# Autodesk Inventor assembly: Sorting Assembly
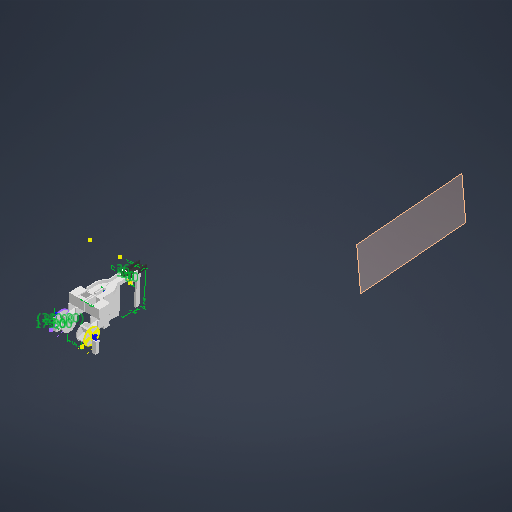
[picture p0: Inventor's stored thumbnail of the model, 512x512]
Saved by Autodesk Inventor 2026.2 (Build 302298000, 298)
## iProperties
Created: 2026-02-23
Part Number: Sorting Assembly
Document SubType Name: Assembly
Designer: danda
Author: danda
## Documents named in this file (17)
- C:\Users\danda\BOM-project\Project\CAD\sorting\Sorting Assembly.iam
- C:\Users\danda\BOM-project\Project\CAD\sorting\stand.ipt
- C:\Users\danda\BOM-project\Project\CAD\sorting\stand2.ipt
- C:\Users\danda\BOM-project\Project\CAD\sorting\inslide.ipt
- C:\Users\danda\BOM-project\Project\CAD\sorting\Towerpro Micro Servo 9g\Towerpro Micro Servo 9g\Towerpro Micro Servo 9g.ipt
- C:\Users\danda\BOM-project\Project\CAD\sorting\motorstand2.ipt
- C:\Users\danda\BOM-project\Project\CAD\sorting\gate2.ipt
- C:\Users\danda\BOM-project\Project\CAD\sorting\wheel.ipt
- C:\Users\danda\BOM-project\Project\CAD\sorting\motorwheelstand.ipt
- C:\Users\danda\BOM-project\Project\CAD\sorting\newmiddle.ipt
- C:\Users\danda\BOM-project\Project\CAD\sorting\leftcollection.ipt
- C:\Users\danda\BOM-project\Project\CAD\sorting\rightcollection.ipt
- C:\Users\danda\Downloads\ir-sensor-7.snapshot.2\Assembly2.iam
- C:\Users\danda\BOM-project\Project\CAD\sorting\wheel_MIR.ipt
- C:\Users\danda\BOM-project\Project\CAD\sorting\Towerpro Micro Servo 9g\Towerpro Micro Servo 9g\Towerpro Micro Servo 9g_MIR.ipt
- C:\Users\danda\BOM-project\Project\CAD\sorting\motorwheelstand_MIR.ipt
- C:\Users\danda\BOM-project\Project\CAD\Not needed\outstorage.ipt
## Components (18 placed, 16 different names)
1. stand:1 — Flush:8, Mate:30, Mate:73, Flush:40, Flush:42
2. stand2:1 — Mate:17, Mate:18, Mate:30, Mate:31, Mate:32, Flush:13
3. inslide:1 — Flush:8, Mate:17, Mate:18, Mate:31, Mate:32, Flush:13, Flush:34, Flush:35, Mate:67, Mate:68, Mate:71, Mate:72
4. motorstand2:1 — Mate:21, Mate:69, Mate:70, Flush:40, Flush:42, Flush:43, Flush:51
5. Towerpro Micro Servo 9g:2 — Mate:21, Mate:69, Mate:70, Insert:5
6. gate2:1 — Insert:5
7. wheel:1 — Insert:3, Mate:79, Flush:48
8. Towerpro Micro Servo 9g:4 — Mate:61, Mate:62, Mate:63, Insert:3
9. motorwheelstand:1 — Mate:61, Mate:62, Mate:63, Flush:50, Flush:51
10. newmiddle:1 — Flush:34, Flush:35, Mate:65, Flush:36, Flush:37, Mate:66, Flush:38, Flush:39, Mate:71, Mate:73, Flush:43
11. leftcollection:1 — Mate:66, Flush:38, Flush:39, Flush:41, Mate:77, Flush:44, Flush:45
12. rightcollection:1 — Mate:65, Flush:36, Flush:37, Flush:46, Flush:47, Mate:78
13. Assembly2:1 [sub-assembly] — Mate:67, Mate:68, Mate:72
14. wheel_MIR:1 — Insert:4, Mate:80, Flush:49
15. Towerpro Micro Servo 9g_MIR:1 — Insert:4, Mate:74, Mate:75, Mate:76
16. motorwheelstand_MIR:1 — Mate:74, Mate:75, Mate:76, Flush:50
17. outstorage:1 — Flush:46, Flush:47, Mate:78, Mate:80, Flush:49
18. outstorage:2 — Mate:77, Flush:44, Flush:45, Mate:79, Flush:48
## Relationships (48: Mate 25, Flush 20, Insert 3)
- Flush:8: stand:1 ↔ inslide:1
- Mate:17: stand2:1 ↔ inslide:1
- Mate:18: stand2:1 ↔ inslide:1
- Mate:21: motorstand2:1 ↔ Towerpro Micro Servo 9g:2
- Mate:30 (85 mm): stand:1 ↔ stand2:1
- Mate:31: stand2:1 ↔ inslide:1
- Mate:32: stand2:1 ↔ inslide:1
- Flush:13: stand2:1 ↔ inslide:1
- Mate:61: Towerpro Micro Servo 9g:4 ↔ motorwheelstand:1
- Mate:62: Towerpro Micro Servo 9g:4 ↔ motorwheelstand:1
- Mate:63: Towerpro Micro Servo 9g:4 ↔ motorwheelstand:1
- Flush:34: inslide:1 ↔ newmiddle:1
- Flush:35: inslide:1 ↔ newmiddle:1
- Mate:65: newmiddle:1 ↔ rightcollection:1
- Flush:36: newmiddle:1 ↔ rightcollection:1
- Flush:37: newmiddle:1 ↔ rightcollection:1
- Mate:66: newmiddle:1 ↔ leftcollection:1
- Flush:38: newmiddle:1 ↔ leftcollection:1
- Flush:39: newmiddle:1 ↔ leftcollection:1
- Mate:67: inslide:1 ↔ Assembly2:1
- Mate:68: inslide:1 ↔ Assembly2:1
- Mate:69: motorstand2:1 ↔ Towerpro Micro Servo 9g:2
- Mate:70: motorstand2:1 ↔ Towerpro Micro Servo 9g:2
- Mate:71: inslide:1 ↔ newmiddle:1
- Mate:72: inslide:1 ↔ Assembly2:1
- Mate:73: stand:1 ↔ newmiddle:1
- Flush:40 (-10 mm): stand:1 ↔ motorstand2:1
- Insert:3: wheel:1 ↔ Towerpro Micro Servo 9g:4
- Flush:41 (2.54 mm): leftcollection:1
- Insert:4: wheel_MIR:1 ↔ Towerpro Micro Servo 9g_MIR:1
- Mate:74: Towerpro Micro Servo 9g_MIR:1 ↔ motorwheelstand_MIR:1
- Mate:75: Towerpro Micro Servo 9g_MIR:1 ↔ motorwheelstand_MIR:1
- Mate:76: Towerpro Micro Servo 9g_MIR:1 ↔ motorwheelstand_MIR:1
- Flush:42: stand:1 ↔ motorstand2:1
- Flush:43 (-30 mm): motorstand2:1 ↔ newmiddle:1
- Mate:77: leftcollection:1 ↔ outstorage:2
- Flush:44: leftcollection:1 ↔ outstorage:2
- Flush:45: leftcollection:1 ↔ outstorage:2
- Flush:46: rightcollection:1 ↔ outstorage:1
- Flush:47: rightcollection:1 ↔ outstorage:1
- Mate:78: rightcollection:1 ↔ outstorage:1
- Mate:79: wheel:1 ↔ outstorage:2
- Mate:80: wheel_MIR:1 ↔ outstorage:1
- Flush:48: wheel:1 ↔ outstorage:2
- Flush:49: wheel_MIR:1 ↔ outstorage:1
- Flush:50: motorwheelstand:1 ↔ motorwheelstand_MIR:1
- Flush:51: motorstand2:1 ↔ motorwheelstand:1
- Insert:5: Towerpro Micro Servo 9g:2 ↔ gate2:1
## Named parameters: Finish3_Area = 163.814, Finish4_Area = 163.814, Finish5_Area = 163.814
note: some values were not read from the file. Shown as the stored number, unit unknown: "Finish3_Area", "Finish4_Area", "Finish5_Area".
